# Autodesk Inventor assembly: Z-AXIS ASSEMBLY
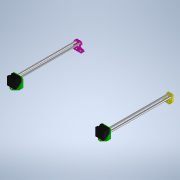
[picture p0: Inventor's stored thumbnail of the model, 180x180]
Saved by Autodesk Inventor 2020.3 (Build 243373010, 373A)
## iProperties
Created: 2019-09-17
Part Number: Z-AXIS ASSEMBLY
Document SubType Name: Assembly
Designer: pepd9
Author: pepd9
## Documents named in this file (10)
- D:\Designs\MK3PRO P1\Z-Axis\Z-AXIS ASSEMBLY.iam
- D:\Designs\MK3PRO P1\Z-Axis\z-axis-bottom-left(P1).ipt
- D:\Designs\MK3PRO P1\Z-Axis\z-axis-bottom-right.ipt
- D:\Designs\MK3PRO P1\Z-Axis\Z-axis_motor_L.ipt
- D:\Designs\MK3PRO P1\Z-Axis\Z-axis_motor_R.ipt
- D:\Designs\MK3PRO P1\Z-Axis\Z-Axis Rod.ipt
- D:\Designs\MK3PRO P1\COMPONENTS\M3 Washer.ipt
- D:\Designs\MK3PRO P1\COMPONENTS\SHCS_M3_10.ipt
- D:\Designs\MK3PRO P1\Z-Axis\z-axis-top-left(P1).ipt
- D:\Designs\MK3PRO P1\Z-Axis\z-axis-top-left(P1)_MIR.ipt
## Components (34 placed, 9 different names)
1. z-axis-bottom-left(P1):1 — Mate:1, Flush:1, Mate:3, Mate:5, Mate:6, Mate:7, Mate:12, Mate:23, Mate:24, Mate:25, Mate:26, Mate:27, Mate:28, Mate:29, Mate:30, Mate:36, Mate:37, Mate:38, Mate:39, Mate:52, Mate:53, Mate:54, Mate:55, Mate:56, Mate:57
2. z-axis-bottom-right:1 — Mate:2, Flush:1, Flush:2, Mate:4, Mate:8, Mate:9, Mate:10, Mate:14, Mate:15, Mate:16, Mate:17, Mate:18, Mate:19, Mate:20, Mate:21, Mate:22, Mate:31, Mate:32, Mate:34, Mate:58, Mate:59, Mate:60, Mate:61, Mate:62, Mate:63
3. Z-axis_motor_L:1 — Mate:5, Mate:6, Mate:7, Mate:11
4. Z-axis_motor_R:1 — Mate:8, Mate:9, Mate:10, Mate:13
5. Z-Axis Rod:1 — Mate:11, Mate:12, Mate:43
6. Z-Axis Rod:2 — Mate:13, Mate:14, Mate:45
7. M3 Washer:1 — Mate:23, Mate:27, Mate:40
8. M3 Washer:2 — Mate:24, Mate:28
9. M3 Washer:3 — Mate:25, Mate:30
10. M3 Washer:4 — Mate:26, Mate:29
11. M3 Washer:5 — Mate:15, Mate:20
12. M3 Washer:6 — Mate:16, Mate:19, Mate:35
13. M3 Washer:7 — Mate:17, Mate:21, Mate:33
14. M3 Washer:8 — Mate:18, Mate:22
15. SHCS_M3_10:1 — Mate:38, Flush:6, Flush:7
16. SHCS_M3_10:2 — Mate:39, Flush:7
17. SHCS_M3_10:3 — Mate:37, Flush:8
18. SHCS_M3_10:4 — Mate:36, Mate:40, Flush:6, Flush:8
19. SHCS_M3_10:5 — Mate:31, Flush:4
20. SHCS_M3_10:6 — Mate:32, Mate:35, Flush:3, Flush:4, Flush:5
21. SHCS_M3_10:7 — Mate:33, Flush:5
22. SHCS_M3_10:8 — Mate:34, Flush:3
23. z-axis-top-left(P1):1 — Mate:41, Mate:43, Mate:44, Flush:9, Mate:49, Mate:50, Mate:51
24. z-axis-top-left(P1)_MIR:1 — Mate:42, Flush:9, Mate:45, Mate:46, Mate:47, Mate:48
25. SHCS_M3_10:9 — Mate:49, Flush:11
26. SHCS_M3_10:10 — Mate:50, Mate:51, Flush:11
27. SHCS_M3_10:11 — Mate:46, Mate:48, Flush:10
28. SHCS_M3_10:12 — Mate:47, Flush:10
29. SHCS_M3_10:13 — Mate:54, Mate:56
30. SHCS_M3_10:14 — Mate:53, Mate:55
31. SHCS_M3_10:15 — Mate:52, Mate:57
32. SHCS_M3_10:16 — Mate:58, Mate:62
33. SHCS_M3_10:17 — Mate:59, Mate:63
34. SHCS_M3_10:18 — Mate:60, Mate:61
## Relationships (74: Mate 63, Flush 11)
- Mate:1: z-axis-bottom-left(P1):1
- Mate:2: z-axis-bottom-right:1
- Flush:1: z-axis-bottom-left(P1):1 ↔ z-axis-bottom-right:1
- Flush:2: z-axis-bottom-right:1
- Mate:3 (-225 mm): z-axis-bottom-left(P1):1
- Mate:4 (225 mm): z-axis-bottom-right:1
- Mate:5: z-axis-bottom-left(P1):1 ↔ Z-axis_motor_L:1
- Mate:6: z-axis-bottom-left(P1):1 ↔ Z-axis_motor_L:1
- Mate:7: z-axis-bottom-left(P1):1 ↔ Z-axis_motor_L:1
- Mate:8: z-axis-bottom-right:1 ↔ Z-axis_motor_R:1
- Mate:9: z-axis-bottom-right:1 ↔ Z-axis_motor_R:1
- Mate:10: z-axis-bottom-right:1 ↔ Z-axis_motor_R:1
- Mate:11: Z-axis_motor_L:1 ↔ Z-Axis Rod:1
- Mate:12: z-axis-bottom-left(P1):1 ↔ Z-Axis Rod:1
- Mate:13: Z-axis_motor_R:1 ↔ Z-Axis Rod:2
- Mate:14: z-axis-bottom-right:1 ↔ Z-Axis Rod:2
- Mate:15: z-axis-bottom-right:1 ↔ M3 Washer:5
- Mate:16: z-axis-bottom-right:1 ↔ M3 Washer:6
- Mate:17: z-axis-bottom-right:1 ↔ M3 Washer:7
- Mate:18: z-axis-bottom-right:1 ↔ M3 Washer:8
- Mate:19: z-axis-bottom-right:1 ↔ M3 Washer:6
- Mate:20: z-axis-bottom-right:1 ↔ M3 Washer:5
- Mate:21: z-axis-bottom-right:1 ↔ M3 Washer:7
- Mate:22: z-axis-bottom-right:1 ↔ M3 Washer:8
- Mate:23: z-axis-bottom-left(P1):1 ↔ M3 Washer:1
- Mate:24: z-axis-bottom-left(P1):1 ↔ M3 Washer:2
- Mate:25: z-axis-bottom-left(P1):1 ↔ M3 Washer:3
- Mate:26: z-axis-bottom-left(P1):1 ↔ M3 Washer:4
- Mate:27: z-axis-bottom-left(P1):1 ↔ M3 Washer:1
- Mate:28: z-axis-bottom-left(P1):1 ↔ M3 Washer:2
- Mate:29: z-axis-bottom-left(P1):1 ↔ M3 Washer:4
- Mate:30: z-axis-bottom-left(P1):1 ↔ M3 Washer:3
- Mate:31: z-axis-bottom-right:1 ↔ SHCS_M3_10:5
- Mate:32: z-axis-bottom-right:1 ↔ SHCS_M3_10:6
- Mate:33: M3 Washer:7 ↔ SHCS_M3_10:7
- Mate:34: z-axis-bottom-right:1 ↔ SHCS_M3_10:8
- Mate:35: M3 Washer:6 ↔ SHCS_M3_10:6
- Flush:3: SHCS_M3_10:6 ↔ SHCS_M3_10:8
- Flush:4: SHCS_M3_10:5 ↔ SHCS_M3_10:6
- Flush:5: SHCS_M3_10:6 ↔ SHCS_M3_10:7
- Mate:36: z-axis-bottom-left(P1):1 ↔ SHCS_M3_10:4
- Mate:37: z-axis-bottom-left(P1):1 ↔ SHCS_M3_10:3
- Mate:38: z-axis-bottom-left(P1):1 ↔ SHCS_M3_10:1
- Mate:39: z-axis-bottom-left(P1):1 ↔ SHCS_M3_10:2
- Mate:40: M3 Washer:1 ↔ SHCS_M3_10:4
- Flush:6: SHCS_M3_10:1 ↔ SHCS_M3_10:4
- Flush:7: SHCS_M3_10:1 ↔ SHCS_M3_10:2
- Flush:8: SHCS_M3_10:3 ↔ SHCS_M3_10:4
- Mate:41: z-axis-top-left(P1):1
- Mate:42: z-axis-top-left(P1)_MIR:1
- Mate:43: Z-Axis Rod:1 ↔ z-axis-top-left(P1):1
- Mate:44 (308 mm): z-axis-top-left(P1):1
- Flush:9: z-axis-top-left(P1):1 ↔ z-axis-top-left(P1)_MIR:1
- Mate:45: Z-Axis Rod:2 ↔ z-axis-top-left(P1)_MIR:1
- Mate:46: z-axis-top-left(P1)_MIR:1 ↔ SHCS_M3_10:11
- Mate:47: z-axis-top-left(P1)_MIR:1 ↔ SHCS_M3_10:12
- Mate:48: z-axis-top-left(P1)_MIR:1 ↔ SHCS_M3_10:11
- Flush:10: SHCS_M3_10:11 ↔ SHCS_M3_10:12
- Mate:49: z-axis-top-left(P1):1 ↔ SHCS_M3_10:9
- Mate:50: z-axis-top-left(P1):1 ↔ SHCS_M3_10:10
- Mate:51: z-axis-top-left(P1):1 ↔ SHCS_M3_10:10
- Flush:11: SHCS_M3_10:9 ↔ SHCS_M3_10:10
- Mate:52: z-axis-bottom-left(P1):1 ↔ SHCS_M3_10:15
- Mate:53: z-axis-bottom-left(P1):1 ↔ SHCS_M3_10:14
- Mate:54: z-axis-bottom-left(P1):1 ↔ SHCS_M3_10:13
- Mate:55: z-axis-bottom-left(P1):1 ↔ SHCS_M3_10:14
- Mate:56: z-axis-bottom-left(P1):1 ↔ SHCS_M3_10:13
- Mate:57: z-axis-bottom-left(P1):1 ↔ SHCS_M3_10:15
- Mate:58: z-axis-bottom-right:1 ↔ SHCS_M3_10:16
- Mate:59: z-axis-bottom-right:1 ↔ SHCS_M3_10:17
- Mate:60: z-axis-bottom-right:1 ↔ SHCS_M3_10:18
- Mate:61: z-axis-bottom-right:1 ↔ SHCS_M3_10:18
- Mate:62: z-axis-bottom-right:1 ↔ SHCS_M3_10:16
- Mate:63: z-axis-bottom-right:1 ↔ SHCS_M3_10:17
